# Autodesk Inventor assembly: Rear_Wheel_Hub_Assembly
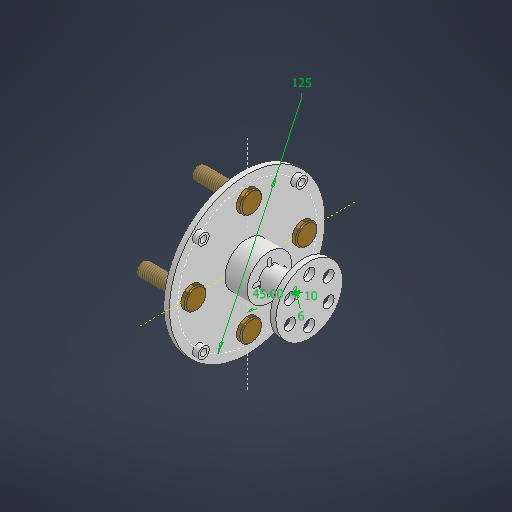
[picture p0: Inventor's stored thumbnail of the model, 512x512]
Saved by Autodesk Inventor 2026.1 (Build 301233000, 233)
## iProperties
Created: 2026-06-12
Part Number: Rear_Wheel_Hub_Assembly
Document SubType Name: Assembly
Designer: share
Author: share
## iProperties of the stored document MemberDocs/xSemtikx4EszrkrsxUhlv4v405e
Created: 2026-06-12
Part Number: Rear_Wheel_Hub_Assembly
Document SubType Name: Assembly
Designer: share
Author: share
## Documents named in this file (13)
- C:\Users\share\OneDrive\Documents\Personal Projects\GOGO Kart\CAD\GOGO_KART_FSAE\Drivetrain\Rear_Wheel_Hub_Assembly.iam
- C:\Users\share\OneDrive\Documents\Personal Projects\GOGO Kart\CAD\GOGO_KART_FSAE\Drivetrain\Hub-CV Adapter.ipt
- C:\Users\share\OneDrive\Documents\Personal Projects\GOGO Kart\CAD\GOGO_KART_FSAE\Drivetrain\Lug Stud M12 X 45.ipt
- C:\Users\share\OneDrive\Documents\Personal Projects\GOGO Kart\CAD\GOGO_KART_FSAE\Drivetrain\Hub.ipt
- C:\Users\share\OneDrive\Documents\Personal Projects\GOGO Kart\CAD\GOGO_KART_FSAE\Suspension\Upright Assembly\Lock Tab.ipt
- C:\Users\share\OneDrive\Documents\Personal Projects\GOGO Kart\CAD\GOGO_KART_FSAE\Suspension\Hardware\90591A171_Zinc-Plated Steel Hex Nut.ipt
- C:\Users\share\OneDrive\Documents\Personal Projects\GOGO Kart\CAD\GOGO_KART_FSAE\Suspension\Upright Assembly\90591A171_Zinc-Plated Steel H.ipt
- C:\Users\share\OneDrive\Documents\Personal Projects\GOGO Kart\CAD\GOGO_KART_FSAE\Drivetrain\Rear_Wheel_Hub_Assembly\AIP\FEA\fh2x0to4g.fins
- C:\Users\share\OneDrive\Documents\Personal Projects\GOGO Kart\CAD\GOGO_KART_FSAE\Drivetrain\Rear_Wheel_Hub_Assembly\AIP\FEA\fh2x0to4g.fsat
- C:\Users\share\OneDrive\Documents\Personal Projects\GOGO Kart\CAD\GOGO_KART_FSAE\Drivetrain\Rear_Wheel_Hub_Assembly\AIP\FEA\fh2x0to4g.ftes
- C:\Users\share\OneDrive\Documents\Personal Projects\GOGO Kart\CAD\GOGO_KART_FSAE\Drivetrain\Rear_Wheel_Hub_Assembly\AIP\FEA\fh2x0to4g.fwiz
- C:\Users\share\OneDrive\Documents\Personal Projects\GOGO Kart\CAD\GOGO_KART_FSAE\Drivetrain\Rear_Wheel_Hub_Assembly\AIP\FEA\fh2x0to74.fmsh
- C:\Users\share\OneDrive\Documents\Personal Projects\GOGO Kart\CAD\GOGO_KART_FSAE\Drivetrain\Rear_Wheel_Hub_Assembly\AIP\FEA\fh2x0to75.fres
## Components (11 placed, 5 different names)
1. Hub-CV Adapter:1 — Flush:1, Mate:1, Flush:2, Flush:3, Flush:4, Insert:9
2. Lug Stud M12 X 45:1 — Insert:2
3. Hub:1 — Insert:1, Insert:2, Insert:3, Insert:4, Flush:1, Mate:1, Insert:5, Insert:6, Mate:2, Insert:7, Mate:3, Insert:8, Mate:4, Insert:9, Insert:10
4. Lug Stud M12 X 45:2 — Insert:4
5. Lug Stud M12 X 45:3 — Insert:3
6. Lug Stud M12 X 45:4 — Insert:1
7. Lock Tab:1 — Insert:5
8. Lock Tab:2 — Insert:6, Mate:2
9. Lock Tab:3 — Insert:7, Mate:3
10. Lock Tab:4 — Insert:8, Mate:4
11. 90591A171_Zinc-Plated Steel Hex Nut:1 — Insert:10
## Relationships (18: Insert 10, Flush 4, Mate 4)
- Insert:1: Hub:1 ↔ Lug Stud M12 X 45:4
- Insert:2: Lug Stud M12 X 45:1 ↔ Hub:1
- Insert:3: Hub:1 ↔ Lug Stud M12 X 45:3
- Insert:4: Hub:1 ↔ Lug Stud M12 X 45:2
- Flush:1: Hub-CV Adapter:1 ↔ Hub:1
- Mate:1: Hub-CV Adapter:1 ↔ Hub:1
- Flush:2: Hub-CV Adapter:1
- Flush:3: Hub-CV Adapter:1
- Flush:4: Hub-CV Adapter:1
- Insert:5: Hub:1 ↔ Lock Tab:1
- Insert:6: Hub:1 ↔ Lock Tab:2
- Mate:2: Hub:1 ↔ Lock Tab:2
- Insert:7: Hub:1 ↔ Lock Tab:3
- Mate:3: Hub:1 ↔ Lock Tab:3
- Insert:8: Hub:1 ↔ Lock Tab:4
- Mate:4: Hub:1 ↔ Lock Tab:4
- Insert:9: Hub-CV Adapter:1 ↔ Hub:1
- Insert:10: Hub:1 ↔ 90591A171_Zinc-Plated Steel Hex Nut:1
## Named parameters: sa_0 = 10000
note: some values were not read from the file. Shown as the stored number, unit unknown: "sa_0".
